# Autodesk Inventor assembly: Bearing_ASM_MIR
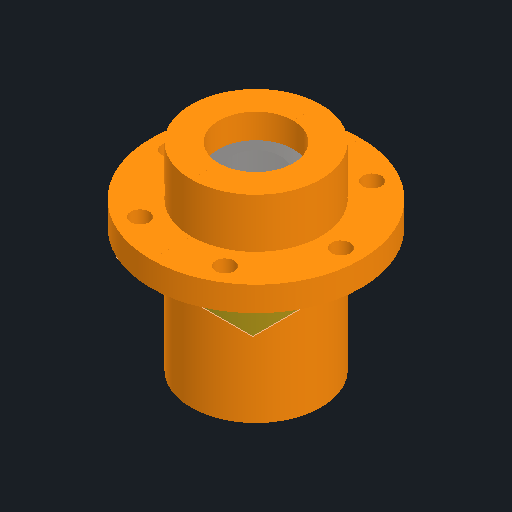
[picture p0: Inventor's stored thumbnail of the model, 512x512]
Saved by Autodesk Inventor 2024.1 (Build 281209000, 209)
## iProperties
Created: 2023-08-04
Part Number: Bearing_ASM_MIR
Document SubType Name: Assembly
Designer: jaege
Author: jaege
## Documents named in this file (3)
- C:\Users\jaege\VUB\Schakel_Ind_Elo\Year_1_Both\BA_Thesis\3D_Files\Lift_V2\Bearing_ASM_MIR.iam
- C:\Users\jaege\VUB\Schakel_Ind_Elo\Year_1_Both\BA_Thesis\3D_Files\Lift_V2\Bearing_Holder_MIR.ipt
- C:\Users\jaege\VUB\Schakel_Ind_Elo\Year_1_Both\BA_Thesis\3D_Files\Lift_V2\LinearBearing_MIR.ipt
## Components (3 placed, 2 different names)
1. Bearing_Holder_MIR:1 — Mate:2, Mate:1, Mate:3
2. LinearBearing_MIR:1 — Mate:2, Mate:1, Mate:4, Mate:5
3. Bearing_Holder_MIR:2 — Mate:3, Mate:4, Mate:5
## Relationships (5: Mate 5)
- Mate:2: Bearing_Holder_MIR:1 ↔ LinearBearing_MIR:1
- Mate:1: Bearing_Holder_MIR:1 ↔ LinearBearing_MIR:1
- Mate:3: Bearing_Holder_MIR:1 ↔ Bearing_Holder_MIR:2
- Mate:4: LinearBearing_MIR:1 ↔ Bearing_Holder_MIR:2
- Mate:5: LinearBearing_MIR:1 ↔ Bearing_Holder_MIR:2
